# Autodesk Inventor assembly: Adrian_Stangeantrieb
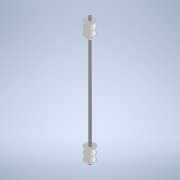
[picture p0: Inventor's stored thumbnail of the model, 180x180]
Saved by Autodesk Inventor 2021 (Build 250183000, 183)
## iProperties
Created: 2022-07-12
Part Number: Adrian_Stangeantrieb
Document SubType Name: Assembly
Designer: adria
Mass: 357.697 g
Surface Area: 534.947 cm^2
Volume: 124.911 cm^3
Density: 2.86362 g/cm^3
Author: adria
## Documents named in this file (6)
- C:\Users\adria\OneDrive - tum.de\G2_Waste-Recycling\CAD\Adrian_Stangeantrieb.iam
- C:\Users\adria\OneDrive - tum.de\G2_Waste-Recycling\CAD\Stange.ipt
- C:\Users\adria\OneDrive - tum.de\G2_Waste-Recycling\CAD\Seil_Rolle_Antrieb_Links.ipt
- C:\Users\adria\OneDrive - tum.de\G2_Waste-Recycling\CAD\Seil_Rolle_Antrieb_Mitte.ipt
- C:\Users\adria\OneDrive - tum.de\G2_Waste-Recycling\CAD\Seil_Rolle_Antrieb_Rechts.ipt
- C:\Users\adria\OneDrive - tum.de\G2_Waste-Recycling\CAD\GT2 Timing Pulley T40.ipt
## Components (8 placed, 5 different names)
1. Stange:1 — Passend:5, Passend:10, Passend:12, Fluchtend:1, Passend:13
2. Seil_Rolle_Antrieb_Links:1 — Passend:2, Passend:3, Passend:11
3. Seil_Rolle_Antrieb_Mitte:1 — Passend:1, Passend:2, Passend:4
4. Seil_Rolle_Antrieb_Rechts:1 — Passend:1, Passend:3, Passend:4, Passend:5, Passend:13
5. Seil_Rolle_Antrieb_Links:2 — Fluchtend:1
6. Seil_Rolle_Antrieb_Mitte:2
7. Seil_Rolle_Antrieb_Rechts:2 — Passend:10
8. GT2 Timing Pulley T40:1 — Passend:11, Passend:12
## Relationships (14: Mate 13, Flush 1)
- Passend:1 [Mate]: Seil_Rolle_Antrieb_Mitte:1 ↔ Seil_Rolle_Antrieb_Rechts:1
- Passend:2 [Mate]: Seil_Rolle_Antrieb_Links:1 ↔ Seil_Rolle_Antrieb_Mitte:1
- Passend:3 [Mate]: Seil_Rolle_Antrieb_Links:1 ↔ Seil_Rolle_Antrieb_Rechts:1
- Passend:4 [Mate]: Seil_Rolle_Antrieb_Mitte:1 ↔ Seil_Rolle_Antrieb_Rechts:1
- Passend:5 [Mate]: Stange:1 ↔ Seil_Rolle_Antrieb_Rechts:1
- [Mate]: Seil_Rolle_Antrieb_Mitte:2 ↔ Seil_Rolle_Antrieb_Rechts:2
- [Mate]: Seil_Rolle_Antrieb_Links:2 ↔ Seil_Rolle_Antrieb_Mitte:2
- [Mate]: Seil_Rolle_Antrieb_Links:2 ↔ Seil_Rolle_Antrieb_Rechts:2
- [Mate]: Seil_Rolle_Antrieb_Mitte:2 ↔ Seil_Rolle_Antrieb_Rechts:2
- Passend:10 [Mate]: Stange:1 ↔ Seil_Rolle_Antrieb_Rechts:2
- Passend:11 [Mate] (1 mm): Seil_Rolle_Antrieb_Links:1 ↔ GT2 Timing Pulley T40:1
- Passend:12 [Mate]: Stange:1 ↔ GT2 Timing Pulley T40:1
- Fluchtend:1 [Flush] (16 mm): Stange:1 ↔ Seil_Rolle_Antrieb_Links:2
- Passend:13 [Mate] (-17 mm): Stange:1 ↔ Seil_Rolle_Antrieb_Rechts:1
## Named parameters: d5_d0 = 0 mm, d6_d1 = 0 mm, d7_d2 = 0 mm, d8_d3 = 0 mm
